# Autodesk Inventor assembly: Platform
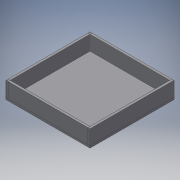
[picture p0: Inventor's stored thumbnail of the model, 180x180]
Saved by Autodesk Inventor 2018 (Build 220112000, 112)
## iProperties
Created: 2019-01-11
Part Number: Platform
Document SubType Name: Assembly
Designer: s-2512711
Author: s-2512711
## Documents named in this file (4)
- \\studenthome\students\S-2512711\GitHub\2019CAD\Drivebase but Calvin is a mad man\Platform.iam
- \\studenthome\students\S-2512711\GitHub\2019CAD\Drivebase but Calvin is a mad man\Platform 29in side.ipt
- \\studenthome\students\S-2512711\GitHub\2019CAD\Drivebase but Calvin is a mad man\Platform 30in side.ipt
- \\studenthome\students\S-2512711\GitHub\2019CAD\Drivebase but Calvin is a mad man\Platform Bottom.ipt
## Components (5 placed, 3 different names)
1. Platform 29in side:1 — Mate:7, Mate:8, Mate:9
2. Platform 29in side:2 — Mate:10, Mate:11, Mate:12
3. Platform 30in side:1 — Mate:4, Mate:5, Mate:6, Mate:9, Mate:12
4. Platform 30in side:2 — Mate:1, Mate:2, Mate:3
5. Platform Bottom:1 — Mate:1, Mate:2, Mate:3, Mate:4, Mate:5, Mate:6, Mate:7, Mate:8, Mate:10, Mate:11
## Relationships (12: Mate 12)
- Mate:1: Platform 30in side:2 ↔ Platform Bottom:1
- Mate:2: Platform 30in side:2 ↔ Platform Bottom:1
- Mate:3: Platform 30in side:2 ↔ Platform Bottom:1
- Mate:4: Platform 30in side:1 ↔ Platform Bottom:1
- Mate:5: Platform 30in side:1 ↔ Platform Bottom:1
- Mate:6: Platform 30in side:1 ↔ Platform Bottom:1
- Mate:7: Platform 29in side:1 ↔ Platform Bottom:1
- Mate:8: Platform 29in side:1 ↔ Platform Bottom:1
- Mate:9: Platform 29in side:1 ↔ Platform 30in side:1
- Mate:10: Platform 29in side:2 ↔ Platform Bottom:1
- Mate:11: Platform 29in side:2 ↔ Platform Bottom:1
- Mate:12: Platform 29in side:2 ↔ Platform 30in side:1
